# Autodesk Inventor assembly: kepala + uv tron board + spacer
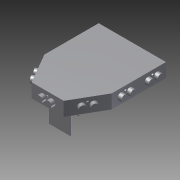
[picture p0: Inventor's stored thumbnail of the model, 180x180]
Saved by Autodesk Inventor 2012 (Build 160160000, 160)
## iProperties
Created: 2013-12-07
Part Number: kepala + uv tron board + spacer
Document SubType Name: Assembly
Designer: Irwan Haryanto
Author: Irwan Haryanto
## Documents named in this file (3)
- D:\Revenant\robot baru 2014\kepala + uv tron board + spacer.iam
- D:\Revenant\robot baru 2014\kepala 120 derajat.ipt
- D:\Revenant\robot baru 2014\spacer 3cm.ipt
## Components (5 placed, 2 different names)
1. kepala 120 derajat:1 — Insert:1, Insert:2, Insert:3, Insert:4
2. spacer 3cm:1 — Insert:4
3. spacer 3cm:2 — Insert:3
4. spacer 3cm:3 — Insert:2
5. spacer 3cm:4 — Insert:1
## Relationships (4: Insert 4)
- Insert:1: kepala 120 derajat:1 ↔ spacer 3cm:4
- Insert:2: kepala 120 derajat:1 ↔ spacer 3cm:3
- Insert:3: kepala 120 derajat:1 ↔ spacer 3cm:2
- Insert:4: kepala 120 derajat:1 ↔ spacer 3cm:1
